# Autodesk Inventor assembly: poleStand
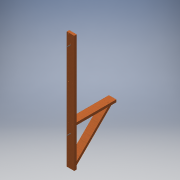
[picture p0: Inventor's stored thumbnail of the model, 180x180]
Saved by Autodesk Inventor 2016 (Build 200138000, 138)
## iProperties
Created: 2013-12-02
Part Number: poleStand
Document SubType Name: Assembly
Designer: Dave
Author: Dave
## Documents named in this file (6)
- C:\Users\krosie\Google Drive\HERA\hera-cad\support\pole\poleStandVertAssy.iam
- C:\Users\krosie\Google Drive\HERA\hera-cad\support\pole\poleStandVert.ipt
- C:\Users\krosie\Google Drive\HERA\hera-cad\support\pole\poleStandHoriz1.ipt
- C:\Users\krosie\Google Drive\HERA\hera-cad\support\pole\poleStand45.ipt
- C:\Users\krosie\Google Drive\HERA\hera-cad\smallParts\washer_3-8.ipt
- C:\Users\krosie\Google Drive\HERA\hera-cad\smallParts\lagBolt_3-8.ipt
## Components (7 placed, 5 different names)
1. poleStandVert:1 — Insert:1, Insert:4, Insert:5, Flush:7, Flush:8, Mate:4
2. poleStand45:1 — Flush:8, Mate:4, Mate:5
3. poleStandHoriz1:1 — Insert:1, Flush:7, Mate:5
4. washer_3-8:2 — Insert:4, Insert:7
5. washer_3-8:3 — Insert:5, Insert:8
6. lagBolt_3-8:1 — Insert:8
7. lagBolt_3-8:2 — Insert:7
## Relationships (9: Insert 5, Flush 2, Mate 2)
- Insert:1: poleStandVert:1 ↔ poleStandHoriz1:1
- Insert:4: poleStandVert:1 ↔ washer_3-8:2
- Insert:5: poleStandVert:1 ↔ washer_3-8:3
- Insert:7: washer_3-8:2 ↔ lagBolt_3-8:2
- Insert:8: washer_3-8:3 ↔ lagBolt_3-8:1
- Flush:7: poleStandVert:1 ↔ poleStandHoriz1:1
- Flush:8: poleStandVert:1 ↔ poleStand45:1
- Mate:4: poleStandVert:1 ↔ poleStand45:1
- Mate:5: poleStand45:1 ↔ poleStandHoriz1:1
